# Autodesk Inventor assembly: Frezowanie_male No.3
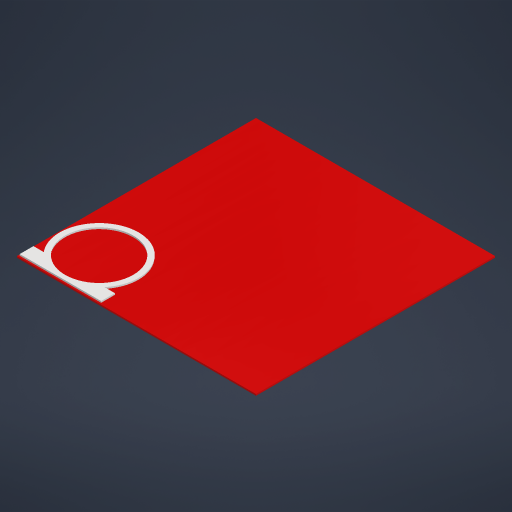
[picture p0: Inventor's stored thumbnail of the model, 512x512]
Saved by Autodesk Inventor 2023 (Build 270158000, 158)
## iProperties
Created: 2023-04-07
Part Number: Frezowanie_male No.3
Document SubType Name: Assembly
Designer: szykr
Author: szykr
## Documents named in this file (3)
- D:\Folder Instalacyjny\GitHub Pliki\Solaris\new model\Frez\Frezowanie_male No.3.iam
- D:\Folder Instalacyjny\GitHub Pliki\Solaris\new model\Frez\Laminat235x235.ipt
- D:\Folder Instalacyjny\GitHub Pliki\Solaris\new model\Frez\Troche Mniejsze(2-31)\Solid17.ipt
## Components (2 placed, 2 different names)
1. Laminat235x235:1 — Mate:1
2. Solid17:1 — Mate:1
## Relationships (1: Mate 1)
- Mate:1: Laminat235x235:1 ↔ Solid17:1
